# Autodesk Inventor assembly: Shed_Area
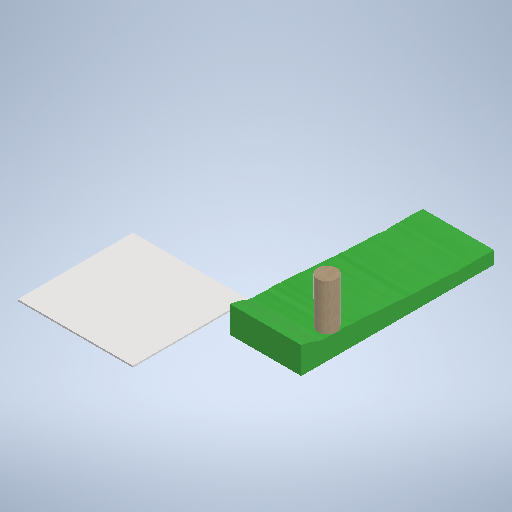
[picture p0: Inventor's stored thumbnail of the model, 512x512]
Saved by Autodesk Inventor 2025 (Build 290162010, 162A)
## iProperties
Created: 2024-08-02
Part Number: Shed_Area
Document SubType Name: Assembly
Designer: Tom
Author: Tom
## Documents named in this file (4)
- C:\Users\Tom\Documents\Inventor\Mobility\Additional_Building\Area_For_Additional_Buildings_With_Piers\Area_For_Additional_Building_With_Foundation_Wall_For_Additional_Building.iam
- C:\Users\Tom\Documents\Inventor\Mobility\Additional_Building\Slab_And_Cross_Section_Of_Foundation_Walls_Of_House.ipt
- C:\Users\Tom\Documents\Inventor\Mobility\Additional_Building\Area_For_Additional_Buildings_With_Piers\Earth_For_Foundation_Wall_For_Additional_Building.ipt
- C:\Users\Tom\Documents\Inventor\Mobility\Additional_Building\Maple_Tree.ipt
## Components (3 placed, 3 different names)
1. Slab_And_Cross_Section_Of_Foundation_Walls_Of_House:1 — Mate:1, Mate:2, Mate:3, Mate:10
2. Earth_For_Foundation_Wall_For_Additional_Building:1 — Mate:1, Mate:2, Mate:3, Tangent:1, Flush:1
3. Maple_Tree:1 — Mate:10, Tangent:1, Flush:1
## Relationships (6: Mate 4, Tangent 1, Flush 1)
- Mate:1 (-1219.2 mm): Slab_And_Cross_Section_Of_Foundation_Walls_Of_House:1 ↔ Earth_For_Foundation_Wall_For_Additional_Building:1
- Mate:2: Slab_And_Cross_Section_Of_Foundation_Walls_Of_House:1 ↔ Earth_For_Foundation_Wall_For_Additional_Building:1
- Mate:3: Slab_And_Cross_Section_Of_Foundation_Walls_Of_House:1 ↔ Earth_For_Foundation_Wall_For_Additional_Building:1
- Mate:10 (1117.6 mm): Slab_And_Cross_Section_Of_Foundation_Walls_Of_House:1 ↔ Maple_Tree:1
- Tangent:1: Earth_For_Foundation_Wall_For_Additional_Building:1 ↔ Maple_Tree:1
- Flush:1: Earth_For_Foundation_Wall_For_Additional_Building:1 ↔ Maple_Tree:1
